# Autodesk Inventor assembly: DC Motor
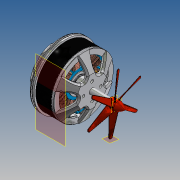
[picture p0: Inventor's stored thumbnail of the model, 180x180]
Saved by Autodesk Inventor 2015 (Build 190159000, 159)
## iProperties
Created: 2016-12-08
Part Number: DC Motor
Document SubType Name: Assembly
Designer: NS
RuleStatus: InUse
BeforeDocSave0: file://iam
Author: NS
## Documents named in this file (8)
- G:\_Vault_ausgecheckt\CAX_Daten\Archiv_SA\2016\DC Motor\DC Motor.iam
- G:\_Vault_ausgecheckt\CAX_Daten\Archiv_SA\2016\DC Motor\stator.ipt
- G:\_Vault_ausgecheckt\CAX_Daten\Archiv_SA\2016\DC Motor\Coil.ipt
- G:\_Vault_ausgecheckt\CAX_Daten\Archiv_SA\2016\DC Motor\Axle.ipt
- G:\_Vault_ausgecheckt\CAX_Daten\Archiv_SA\2016\DC Motor\Bell.ipt
- G:\_Vault_ausgecheckt\CAX_Daten\Archiv_SA\2016\DC Motor\Fan.ipt
- G:\_Vault_ausgecheckt\Bibliotheken\Content Center Files\en-US\DIN BEARING(1)\DIN 625 SKF - SKF 618_5.ipt
- G:\_Vault_ausgecheckt\CAX_Daten\Archiv_SA\2016\DC Motor\Circlip.ipt
## Components (9 placed, 7 different names)
1. stator:1 — Mate:1, Mate:2, Flush:1, Mate:3, Mate:4, Mate:5, Mate:7, Flush:2, Mate:10, Mate:11, Mate:12, Mate:13
2. Coil:1 — Mate:3, Mate:4
3. Axle:1 — Mate:5, Mate:6, Flush:2, Mate:8, Mate:9, Mate:15, Mate:16
4. Bell:1 — Mate:6, Mate:7
5. Fan:1 — Mate:8, Mate:9
6. DIN 625 SKF 618/5:1 — Mate:10, Mate:11, Mate:17
7. DIN 625 SKF 618/5:2 — Mate:12, Mate:13, Mate:14
8. Circlip:1 — Mate:14, Mate:15
9. Circlip:2 — Mate:16, Mate:17
## Relationships (19: Mate 17, Flush 2)
- Mate:1: stator:1
- Mate:2: stator:1
- Flush:1: stator:1
- Mate:3: stator:1 ↔ Coil:1
- Mate:4: stator:1 ↔ Coil:1
- Mate:5: stator:1 ↔ Axle:1
- Mate:6: Axle:1 ↔ Bell:1
- Mate:7: stator:1 ↔ Bell:1
- Flush:2: stator:1 ↔ Axle:1
- Mate:8: Axle:1 ↔ Fan:1
- Mate:9 (-3 mm): Axle:1 ↔ Fan:1
- Mate:10: stator:1 ↔ DIN 625 SKF 618/5:1
- Mate:11: stator:1 ↔ DIN 625 SKF 618/5:1
- Mate:12: stator:1 ↔ DIN 625 SKF 618/5:2
- Mate:13: stator:1 ↔ DIN 625 SKF 618/5:2
- Mate:14: DIN 625 SKF 618/5:2 ↔ Circlip:1
- Mate:15: Axle:1 ↔ Circlip:1
- Mate:16: Axle:1 ↔ Circlip:2
- Mate:17: DIN 625 SKF 618/5:1 ↔ Circlip:2
